# Autodesk Inventor assembly: shoot+intake
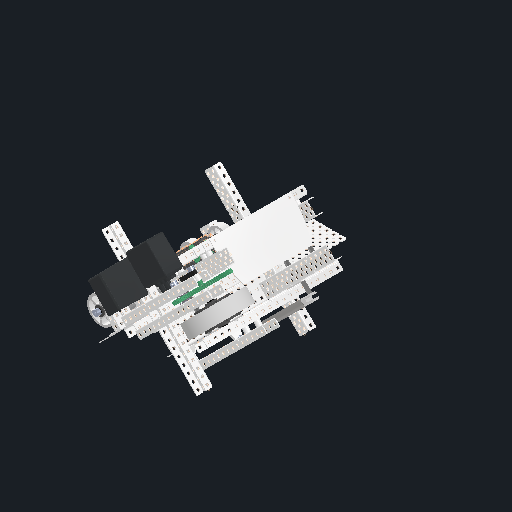
[picture p0: Inventor's stored thumbnail of the model, 512x512]
Saved by Autodesk Inventor 2023 (Build 270158000, 158)
## iProperties
Created: 2023-04-09
Part Number: shoot+intake
Document SubType Name: Assembly
Designer: Windows Macbook
Author: Windows Macbook
## Documents named in this file (39)
- C:\Users\Windows Macbook\Desktop\VRC-SPIN-UP\Inventor\Assembly\Worlds\shoot+intake.iam
- C:\Users\Windows Macbook\Desktop\VRC-SPIN-UP\Inventor\Structure\Standoff\Standoff .50.ipt
- C:\Users\Windows Macbook\Desktop\VRC-SPIN-UP\Inventor\Structure\Standoff.ipt
- C:\Users\Windows Macbook\Desktop\VRC-SPIN-UP\Inventor\Structure\Plate\Steel\Steel Plate 1x8.ipt
- C:\Users\Windows Macbook\Desktop\VRC-SPIN-UP\Inventor\Structure\C Channel\Aluminum 1x2x1\Alu C 1x2x1x14.ipt
- C:\Users\Windows Macbook\Desktop\VRC-SPIN-UP\Inventor\Structure\C Channel\Aluminum 1x2x1\Alu C 1x2x1x20.ipt
- C:\Users\Windows Macbook\Desktop\VRC-SPIN-UP\Inventor\Structure\Plate\Aluminum\Alu Plate 5x25.ipt
- C:\Users\Windows Macbook\Desktop\VRC-SPIN-UP\Inventor\Assembly\Worlds\intake.ipt
- C:\Users\Windows Macbook\Desktop\VRC-SPIN-UP\Inventor\Structure\C Channel\Aluminum 1x2x1\Alu C 1x2x1x25.ipt
- C:\Users\Windows Macbook\Desktop\VRC-SPIN-UP\Inventor\Structure\C Channel\Aluminum 1x2x1\Alu C 1x2x1x15.ipt
- C:\Users\Windows Macbook\Desktop\VRC-SPIN-UP\Inventor\Motion\Spacers\Spacer Nylon .313 OD\NSpacer .313 OD x .250.ipt
- C:\Users\Windows Macbook\Desktop\VRC-SPIN-UP\Inventor\Motion\Spacers\Spacer Nylon .313 OD.ipt
- C:\Users\Windows Macbook\Desktop\VRC-SPIN-UP\Inventor\Motion\Wheels\Flex Wheels\4 Flex, LS.iam
- C:\Users\Windows Macbook\Desktop\VRC-SPIN-UP\Inventor\Motion\Reference Files\Shaft Collar Metal.ipt
- C:\Users\Windows Macbook\Desktop\VRC-SPIN-UP\Inventor\Motion\Shaft LS\Bearing Flat.ipt
- C:\Users\Windows Macbook\Desktop\VRC-SPIN-UP\Inventor\Structure\Standoff\Standoff 2.50.ipt
- C:\Users\Windows Macbook\Desktop\VRC-SPIN-UP\Inventor\Motion\Spacers\Spacer Nylon .313 OD\NSpacer .313 OD x .375.ipt
- C:\Users\Windows Macbook\Desktop\VRC-SPIN-UP\Inventor\Motion\Spacers\Spacer Nylon .313 OD\NSpacer .313 OD x .500.ipt
- C:\Users\Windows Macbook\Desktop\VRC-SPIN-UP\Inventor\Structure\Gussets\90 Angle Gusset.ipt
- C:\Users\Windows Macbook\Desktop\VRC-SPIN-UP\Inventor\Assembly\Worlds\shoot.ipt
- C:\Users\Windows Macbook\Desktop\VRC-SPIN-UP\Inventor\Structure\Standoff\Standoff 1.50.ipt
- C:\Users\Windows Macbook\Desktop\VRC-SPIN-UP\Inventor\Electronics\V5 Simple Motor.ipt
- C:\Users\Windows Macbook\Desktop\VRC-SPIN-UP\Inventor\Structure\C Channel\Aluminum 1x2x1\Alu C 1x2x1x5.ipt
- C:\Users\Windows Macbook\Desktop\VRC-SPIN-UP\Inventor\Motion\Shaft LS\Shaft LS.ipt
- C:\Users\Windows Macbook\Desktop\VRC-SPIN-UP\Inventor\Motion\Wheels\Flex Wheels\1.625 Flex, LS.iam
- C:\Users\Windows Macbook\Desktop\VRC-SPIN-UP\Inventor\Motion\Wheels\Flex Wheels\2 Flex, LS.iam
- C:\Users\Windows Macbook\Desktop\VRC-SPIN-UP\Inventor\Motion\Sprockets\9P Sprocket\9P 6T Sprocket, Square.iam
- C:\Users\Windows Macbook\Desktop\VRC-SPIN-UP\Inventor\Motion\Sprockets\9P Sprocket.iam
- C:\Users\Windows Macbook\Desktop\VRC-SPIN-UP\Inventor\Motion\Shaft LS\Shaft LS\Shaft LS 5.5.ipt
- C:\Users\Windows Macbook\Desktop\VRC-SPIN-UP\Inventor\Motion\Shaft LS\Shaft LS\Shaft LS 8.5.ipt
- C:\Users\Windows Macbook\Desktop\VRC-SPIN-UP\Inventor\Assembly\Worlds\shoot2.ipt
- C:\Users\Windows Macbook\Desktop\VRC-SPIN-UP\Inventor\Motion\Gears\LS 84T Gear.ipt
- C:\Users\Windows Macbook\Desktop\VRC-SPIN-UP\Inventor\Motion\Gears\HS Gear\HS 12T Gear, Square.iam
- C:\Users\Windows Macbook\Desktop\VRC-SPIN-UP\Inventor\Motion\Gears\HS Gear.iam
- C:\Users\Windows Macbook\Desktop\VRC-SPIN-UP\Inventor\Motion\Spacers\Spacer Nylon .313 OD\NSpacer .313 OD x .125.ipt
- C:\Users\Windows Macbook\Desktop\VRC-SPIN-UP\Inventor\Motion\Chain Generator 9P\Chain Generator 9P (06x06x3.5).ipt
- C:\Users\Windows Macbook\Desktop\VRC-SPIN-UP\Inventor\Motion\Chain Generator 9P\Chain Generator 9P (06x06x3).ipt
- C:\Users\Windows Macbook\Desktop\VRC-SPIN-UP\Inventor\Structure\C Channel\Aluminum 1x3x1\Alu C 1x3x1x15.ipt
- C:\Users\Windows Macbook\Desktop\VRC-SPIN-UP\Inventor\Assembly\Worlds\indexer.iam
## Components (113 placed, 33 different names)
1. Alu Plate 5x25:1 — Angle:1
2. Alu C 1x2x1x14:3 — Insert:39, Insert:67, Angle:2, Insert:72, Insert:73, Insert:76, Insert:77
3. intake:1 — Angle:1, Insert:5, Insert:6, Insert:7, Insert:8, Insert:17, Insert:18
4. Alu C 1x2x1x25:1 — Insert:5, Insert:6, Insert:10, Insert:19, Insert:20, Insert:25, Insert:26, Insert:172, Insert:173, Angle:3
5. Alu C 1x2x1x25:2 — Insert:7, Insert:8, Insert:21, Insert:22, Insert:29, Insert:30, Insert:31, Insert:32, Insert:175, Insert:176
6. Alu C 1x2x1x20:2 — Insert:12, Insert:15, Insert:16, Insert:49, Insert:69, Insert:79, Insert:80, Insert:125, Insert:131, Insert:149, Insert:151, Insert:152, Insert:167
7. Standoff .50:5 — Insert:10, Insert:12
8. Alu C 1x2x1x15:1 — Insert:15, Insert:16, Insert:177, Insert:178
9. Alu C 1x2x1x15:2 — Insert:23, Insert:24, Insert:140, Insert:141
10. Alu C 1x2x1x15:3 — Insert:17, Insert:18
11. Alu C 1x2x1x15:4 — Insert:27, Insert:28
12. NSpacer .313 OD x .250:1 — Insert:20, Insert:24
13. NSpacer .313 OD x .250:2 — Insert:21
14. NSpacer .313 OD x .250:3 — Insert:25, Insert:28
15. NSpacer .313 OD x .250:4 — Insert:29
16. NSpacer .313 OD x .250:5 — Insert:26, Insert:27
17. NSpacer .313 OD x .250:6 — Insert:30
18. NSpacer .313 OD x .250:7 — Insert:19, Insert:23
19. NSpacer .313 OD x .250:8 — Insert:22
20. Standoff .50:7 — Insert:31, Insert:34
21. Standoff .50:8 — Insert:32, Insert:33
22. Alu C 1x2x1x20:3 — Insert:33, Insert:34, Insert:68, Angle:2, Insert:119, Insert:120
23. Alu C 1x2x1x15:5 — Insert:49, Insert:53, Insert:54, Insert:69
24. Standoff .50:9 — Insert:39, Insert:68
25. Standoff .50:10 — Insert:67
26. Alu C 1x2x1x20:5 — Insert:74, Insert:75
27. 4 Flex, LS:1 [sub-assembly] — Insert:142
28. Shaft Collar Metal:1
29. Bearing Flat:1
30. NSpacer .313 OD x .375:9 — Insert:51, Insert:54
31. NSpacer .313 OD x .500:10 — Insert:51
32. NSpacer .313 OD x .375:11 — Insert:53
33. NSpacer .313 OD x .500:12
34. 90 Angle Gusset:1 — Insert:70, Insert:71
35. shoot:1 — Insert:70, Insert:71, Insert:72, Insert:73, Insert:74, Insert:75, Insert:78, Insert:186, Angle:4
36. Standoff 1.50:11 — Insert:76
37. Standoff 1.50:12 — Insert:77
38. Standoff 2.50:14 — Insert:78
39. V5 Simple Motor:1 — Insert:79, Insert:80
40. Standoff .50:15 — Insert:173
41. Standoff .50:16 — Insert:172, Insert:174
42. Standoff .50:17 — Insert:85, Insert:175
43. Standoff .50:18 — Insert:86, Insert:176
44. Alu C 1x2x1x5:1 — Insert:85, Insert:86, Insert:117, Insert:121, Insert:122
45. Alu C 1x2x1x5:2 — Insert:123, Insert:124, Insert:129, Insert:174, Angle:3
46. Steel Plate 1x8:1
47. 1.625 Flex, LS:1 [sub-assembly]
48. Shaft Collar Metal:2 — Insert:117
49. 2 Flex, LS:1 [sub-assembly]
50. Shaft Collar Metal:3
51. Bearing Flat:2
52. Shaft Collar Metal:4 — Flush:1, Rigid:1
53. Steel Plate 1x8:2
54. 1.625 Flex, LS:2 [sub-assembly]
55. 2 Flex, LS:2 [sub-assembly]
56. Shaft Collar Metal:5 — Insert:130
57. Bearing Flat:3
58. Shaft Collar Metal:6 — Flush:2, Rigid:2
59. Shaft Collar Metal:7 — Insert:129
60. 2 Flex, LS:3 [sub-assembly]
61. Shaft Collar Metal:8
62. Shaft Collar Metal:9
63. 9P 6T Sprocket, Square:1 [sub-assembly] — Insert:139
64. 9P 6T Sprocket, Square:2 [sub-assembly] — Insert:137
65. Shaft Collar Metal:10
66. Shaft Collar Metal:11
67. NSpacer .313 OD x .500:13
68. NSpacer .313 OD x .500:14
69. Bearing Flat:4 — Insert:119, Insert:120, Insert:128
70. Bearing Flat:5 — Insert:121, Insert:122, Insert:127
71. Bearing Flat:6 — Insert:123, Insert:124, Insert:126
72. Shaft Collar Metal:12 — Insert:127, Rigid:3
73. Shaft Collar Metal:13 — Insert:126
74. Shaft Collar Metal:14 — Insert:128, Rigid:4
75. Shaft Collar Metal:15 — Insert:125
76. Shaft LS 8.5:1 — Rigid:3
77. Shaft LS 8.5:2 — Rigid:4
78. Shaft LS 5.5:3 — Flush:1, Rigid:1, Flush:2, Rigid:2
79. 9P 6T Sprocket, Square:3 [sub-assembly] — Insert:130
80. 9P 6T Sprocket, Square:4 [sub-assembly] — Insert:131, Insert:132, Insert:133
81. NSpacer .313 OD x .375:15 — Insert:132, Insert:134
82. 9P 6T Sprocket, Square:5 [sub-assembly] — Insert:134, Insert:135
83. Shaft Collar Metal:16 — Insert:133, Insert:183
84. Shaft Collar Metal:17 — Insert:135, Insert:185
85. Chain Generator 9P (06x06x3):1 — Insert:139
86. Chain Generator 9P (06x06x3.5):1 — Insert:137
87. shoot2:1 — Insert:140, Insert:141
88. NSpacer .313 OD x .500:16 — Insert:142
89. LS 84T Gear:1 — Insert:145, Insert:156
90. HS 12T Gear, Square:1 [sub-assembly] — Insert:157
91. NSpacer .313 OD x .125:17 — Insert:145
92. Alu C 1x2x1x15:6 — Insert:161, Insert:163, Insert:164, Insert:168, Insert:169, Insert:170, Insert:171
93. Standoff .50:21 — Insert:149, Insert:168
94. Standoff .50:22 — Insert:167, Insert:169
95. Standoff .50:23 — Insert:151, Insert:154
96. Standoff .50:24 — Insert:152, Insert:155
97. Alu C 1x2x1x15:7 — Insert:154, Insert:155, Insert:158, Insert:159
98. NSpacer .313 OD x .375:18 — Insert:156
99. NSpacer .313 OD x .500:19 — Insert:157
100. Shaft Collar Metal:19 — Insert:160
101. Bearing Flat:7 — Insert:158, Insert:159, Insert:160
102. Shaft Collar Metal:20 — Insert:161
103. Shaft Collar Metal:21
104. Bearing Flat:8 — Insert:163, Insert:164
105. V5 Simple Motor:2 — Insert:170, Insert:171
106. Alu C 1x3x1x15:1 — Insert:177, Insert:178
107. 1.625 Flex, LS:3 [sub-assembly] — Insert:184
108. Shaft Collar Metal:22
109. Shaft Collar Metal:23
110. 1.625 Flex, LS:4 [sub-assembly]
111. Shaft Collar Metal:24 — Insert:183
112. Shaft Collar Metal:25 — Insert:184, Insert:185
113. indexer:1 [sub-assembly] — Insert:186, Angle:4
## Relationships (142: Insert 132, Angle 4, WeldJoint 4, Flush 2)
- Angle:1 (135 deg): Alu Plate 5x25:1 ↔ intake:1
- Insert:5: intake:1 ↔ Alu C 1x2x1x25:1
- Insert:6: intake:1 ↔ Alu C 1x2x1x25:1
- Insert:7: intake:1 ↔ Alu C 1x2x1x25:2
- Insert:8: intake:1 ↔ Alu C 1x2x1x25:2
- Insert:10: Alu C 1x2x1x25:1 ↔ Standoff .50:5
- Insert:12: Alu C 1x2x1x20:2 ↔ Standoff .50:5
- Insert:15: Alu C 1x2x1x20:2 ↔ Alu C 1x2x1x15:1
- Insert:16: Alu C 1x2x1x20:2 ↔ Alu C 1x2x1x15:1
- Insert:17: intake:1 ↔ Alu C 1x2x1x15:3
- Insert:18: intake:1 ↔ Alu C 1x2x1x15:3
- Insert:19: Alu C 1x2x1x25:1 ↔ NSpacer .313 OD x .250:7
- Insert:20: Alu C 1x2x1x25:1 ↔ NSpacer .313 OD x .250:1
- Insert:21: Alu C 1x2x1x25:2 ↔ NSpacer .313 OD x .250:2
- Insert:22: Alu C 1x2x1x25:2 ↔ NSpacer .313 OD x .250:8
- Insert:23: Alu C 1x2x1x15:2 ↔ NSpacer .313 OD x .250:7
- Insert:24: Alu C 1x2x1x15:2 ↔ NSpacer .313 OD x .250:1
- Insert:25: Alu C 1x2x1x25:1 ↔ NSpacer .313 OD x .250:3
- Insert:26: Alu C 1x2x1x25:1 ↔ NSpacer .313 OD x .250:5
- Insert:27: Alu C 1x2x1x15:4 ↔ NSpacer .313 OD x .250:5
- Insert:28: Alu C 1x2x1x15:4 ↔ NSpacer .313 OD x .250:3
- Insert:29: Alu C 1x2x1x25:2 ↔ NSpacer .313 OD x .250:4
- Insert:30: Alu C 1x2x1x25:2 ↔ NSpacer .313 OD x .250:6
- Insert:31: Alu C 1x2x1x25:2 ↔ Standoff .50:7
- Insert:32: Alu C 1x2x1x25:2 ↔ Standoff .50:8
- Insert:33: Standoff .50:8 ↔ Alu C 1x2x1x20:3
- Insert:34: Standoff .50:7 ↔ Alu C 1x2x1x20:3
- Insert:39: Alu C 1x2x1x14:3 ↔ Standoff .50:9
- [Insert]: Alu C 1x2x1x20:5 ↔ 4 Flex, LS:1
- [Insert]: Shaft Collar Metal:1 ↔ Bearing Flat:1
- [Insert]: Alu C 1x2x1x20:5 ↔ Bearing Flat:1
- [Insert]: Alu C 1x2x1x20:5 ↔ Bearing Flat:1
- Insert:49: Alu C 1x2x1x20:2 ↔ Alu C 1x2x1x15:5
- Insert:51: NSpacer .313 OD x .375:9 ↔ NSpacer .313 OD x .500:10
- [Insert]: NSpacer .313 OD x .375:11 ↔ NSpacer .313 OD x .500:12
- Insert:53: Alu C 1x2x1x15:5 ↔ NSpacer .313 OD x .375:11
- Insert:54: Alu C 1x2x1x15:5 ↔ NSpacer .313 OD x .375:9
- Insert:67: Alu C 1x2x1x14:3 ↔ Standoff .50:10
- Insert:68: Alu C 1x2x1x20:3 ↔ Standoff .50:9
- Angle:2 (-90 deg): Alu C 1x2x1x14:3 ↔ Alu C 1x2x1x20:3
- Insert:69: Alu C 1x2x1x20:2 ↔ Alu C 1x2x1x15:5
- Insert:70: 90 Angle Gusset:1 ↔ shoot:1
- Insert:71: 90 Angle Gusset:1 ↔ shoot:1
- Insert:72: Alu C 1x2x1x14:3 ↔ shoot:1
- Insert:73: Alu C 1x2x1x14:3 ↔ shoot:1
- Insert:74: Alu C 1x2x1x20:5 ↔ shoot:1
- Insert:75: Alu C 1x2x1x20:5 ↔ shoot:1
- Insert:76: Alu C 1x2x1x14:3 ↔ Standoff 1.50:11
- Insert:77: Alu C 1x2x1x14:3 ↔ Standoff 1.50:12
- Insert:78: shoot:1 ↔ Standoff 2.50:14
- Insert:79: Alu C 1x2x1x20:2 ↔ V5 Simple Motor:1
- Insert:80: Alu C 1x2x1x20:2 ↔ V5 Simple Motor:1
- Insert:85: Standoff .50:17 ↔ Alu C 1x2x1x5:1
- Insert:86: Standoff .50:18 ↔ Alu C 1x2x1x5:1
- [Insert]: 1.625 Flex, LS:1 ↔ Shaft Collar Metal:2
- [Insert]: Steel Plate 1x8:1 ↔ 2 Flex, LS:1
- [Insert]: Steel Plate 1x8:1 ↔ Bearing Flat:2
- [Insert]: Steel Plate 1x8:1 ↔ Bearing Flat:2
- [Insert]: Shaft Collar Metal:3 ↔ Bearing Flat:2
- [Insert]: Steel Plate 1x8:1 ↔ 1.625 Flex, LS:1
- [Insert]: 2 Flex, LS:1 ↔ Shaft Collar Metal:4
- [Insert]: Steel Plate 1x8:2 ↔ 2 Flex, LS:2
- [Insert]: Steel Plate 1x8:2 ↔ Bearing Flat:3
- [Insert]: Steel Plate 1x8:2 ↔ Bearing Flat:3
- [Insert]: Shaft Collar Metal:5 ↔ Bearing Flat:3
- [Insert]: Steel Plate 1x8:2 ↔ 1.625 Flex, LS:2
- [Insert]: 2 Flex, LS:2 ↔ Shaft Collar Metal:6
- [Insert]: 1.625 Flex, LS:2 ↔ Shaft Collar Metal:7
- [Insert]: 2 Flex, LS:3 ↔ Shaft Collar Metal:9
- [Insert]: 2 Flex, LS:3 ↔ Shaft Collar Metal:8
- [Insert] (12.7 mm): Shaft Collar Metal:3 ↔ Shaft Collar Metal:9
- [Insert]: Steel Plate 1x8:2 ↔ NSpacer .313 OD x .500:13
- [Insert]: Steel Plate 1x8:1 ↔ NSpacer .313 OD x .500:14
- [Insert]: 9P 6T Sprocket, Square:1 ↔ NSpacer .313 OD x .500:14
- [Insert]: 9P 6T Sprocket, Square:2 ↔ NSpacer .313 OD x .500:13
- [Insert]: 9P 6T Sprocket, Square:2 ↔ Shaft Collar Metal:11
- [Insert]: 9P 6T Sprocket, Square:1 ↔ Shaft Collar Metal:10
- Insert:117 (19.05 mm): Alu C 1x2x1x5:1 ↔ Shaft Collar Metal:2
- Insert:119: Alu C 1x2x1x20:3 ↔ Bearing Flat:4
- Insert:120: Alu C 1x2x1x20:3 ↔ Bearing Flat:4
- Insert:121: Alu C 1x2x1x5:1 ↔ Bearing Flat:5
- Insert:122: Alu C 1x2x1x5:1 ↔ Bearing Flat:5
- Insert:123: Alu C 1x2x1x5:2 ↔ Bearing Flat:6
- Insert:124: Alu C 1x2x1x5:2 ↔ Bearing Flat:6
- Insert:125: Alu C 1x2x1x20:2 ↔ Shaft Collar Metal:15
- Insert:126: Bearing Flat:6 ↔ Shaft Collar Metal:13
- Insert:127: Bearing Flat:5 ↔ Shaft Collar Metal:12
- Insert:128: Bearing Flat:4 ↔ Shaft Collar Metal:14
- Flush:1: Shaft Collar Metal:4 ↔ Shaft LS 5.5:3
- Rigid:1 [WeldJoint]: Shaft Collar Metal:4 ↔ Shaft LS 5.5:3
- Flush:2: Shaft Collar Metal:6 ↔ Shaft LS 5.5:3
- Rigid:2 [WeldJoint]: Shaft Collar Metal:6 ↔ Shaft LS 5.5:3
- Insert:129 (19.05 mm): Alu C 1x2x1x5:2 ↔ Shaft Collar Metal:7
- Rigid:3 [WeldJoint] (4.7625 mm): Shaft Collar Metal:12 ↔ Shaft LS 8.5:1
- Rigid:4 [WeldJoint]: Shaft Collar Metal:14 ↔ Shaft LS 8.5:2
- Insert:130: Shaft Collar Metal:5 ↔ 9P 6T Sprocket, Square:3
- Insert:131 (82.2325 mm): Alu C 1x2x1x20:2 ↔ 9P 6T Sprocket, Square:4
- Insert:132: 9P 6T Sprocket, Square:4 ↔ NSpacer .313 OD x .375:15
- Insert:133: 9P 6T Sprocket, Square:4 ↔ Shaft Collar Metal:16
- Insert:134: NSpacer .313 OD x .375:15 ↔ 9P 6T Sprocket, Square:5
- Insert:135: 9P 6T Sprocket, Square:5 ↔ Shaft Collar Metal:17
- Insert:137 (-1.27 mm): 9P 6T Sprocket, Square:2 ↔ Chain Generator 9P (06x06x3.5):1
- Insert:139 (1.27 mm): 9P 6T Sprocket, Square:1 ↔ Chain Generator 9P (06x06x3):1
- Insert:140: Alu C 1x2x1x15:2 ↔ shoot2:1
- Insert:141: Alu C 1x2x1x15:2 ↔ shoot2:1
- Insert:142: 4 Flex, LS:1 ↔ NSpacer .313 OD x .500:16
- Insert:145: LS 84T Gear:1 ↔ NSpacer .313 OD x .125:17
- Insert:149: Alu C 1x2x1x20:2 ↔ Standoff .50:21
- Insert:151: Alu C 1x2x1x20:2 ↔ Standoff .50:23
- Insert:152: Alu C 1x2x1x20:2 ↔ Standoff .50:24
- Insert:154: Standoff .50:23 ↔ Alu C 1x2x1x15:7
- Insert:155: Standoff .50:24 ↔ Alu C 1x2x1x15:7
- Insert:156: LS 84T Gear:1 ↔ NSpacer .313 OD x .375:18
- Insert:157: HS 12T Gear, Square:1 ↔ NSpacer .313 OD x .500:19
- Insert:158: Alu C 1x2x1x15:7 ↔ Bearing Flat:7
- Insert:159: Alu C 1x2x1x15:7 ↔ Bearing Flat:7
- Insert:160: Shaft Collar Metal:19 ↔ Bearing Flat:7
- Insert:161: Alu C 1x2x1x15:6 ↔ Shaft Collar Metal:20
- [Insert]: Shaft Collar Metal:21 ↔ Bearing Flat:8
- Insert:163: Alu C 1x2x1x15:6 ↔ Bearing Flat:8
- Insert:164: Alu C 1x2x1x15:6 ↔ Bearing Flat:8
- Insert:167: Alu C 1x2x1x20:2 ↔ Standoff .50:22
- Insert:168: Alu C 1x2x1x15:6 ↔ Standoff .50:21
- Insert:169: Alu C 1x2x1x15:6 ↔ Standoff .50:22
- Insert:170: Alu C 1x2x1x15:6 ↔ V5 Simple Motor:2
- Insert:171: Alu C 1x2x1x15:6 ↔ V5 Simple Motor:2
- Insert:172: Alu C 1x2x1x25:1 ↔ Standoff .50:16
- Insert:173: Alu C 1x2x1x25:1 ↔ Standoff .50:15
- Insert:174: Standoff .50:16 ↔ Alu C 1x2x1x5:2
- Angle:3 (0 deg): Alu C 1x2x1x25:1 ↔ Alu C 1x2x1x5:2
- Insert:175: Alu C 1x2x1x25:2 ↔ Standoff .50:17
- Insert:176: Alu C 1x2x1x25:2 ↔ Standoff .50:18
- Insert:177: Alu C 1x2x1x15:1 ↔ Alu C 1x3x1x15:1
- Insert:178: Alu C 1x2x1x15:1 ↔ Alu C 1x3x1x15:1
- [Insert]: 1.625 Flex, LS:3 ↔ Shaft Collar Metal:22
- [Insert]: 1.625 Flex, LS:4 ↔ Shaft Collar Metal:24
- [Insert]: Shaft Collar Metal:23 ↔ 1.625 Flex, LS:4
- Insert:183 (25.4 mm): Shaft Collar Metal:16 ↔ Shaft Collar Metal:24
- Insert:184: 1.625 Flex, LS:3 ↔ Shaft Collar Metal:25
- Insert:185: Shaft Collar Metal:17 ↔ Shaft Collar Metal:25
- Insert:186: shoot:1 ↔ indexer:1
- Angle:4 (0 deg): shoot:1 ↔ indexer:1
## Named parameters: d58_d57 = 0 mm, d108_d89 = 0 mm, d109_d90 = 0 mm, d112_d93 = 0 mm, d113_d94 = 0 mm, d117_d87 = 0 mm, d118_d88 = 12.7 mm, d119_d55 = 0 mm, d120_d57 = 0 mm, d122_d59 = 0 mm, d123_d60 = 0 mm, d65_d57 = 0 mm, d66_d58 = 0 mm, d67_d59 = 0 mm, d68_d60 = 0 mm, d69_d61 = 0 mm, d195_d128 = 0 mm, d217_d119_d55 = 0 mm, d219_d217_d119_d55 = 0 mm, d220_d218 = 0 mm
